# Autodesk Inventor assembly: 足全体_temp
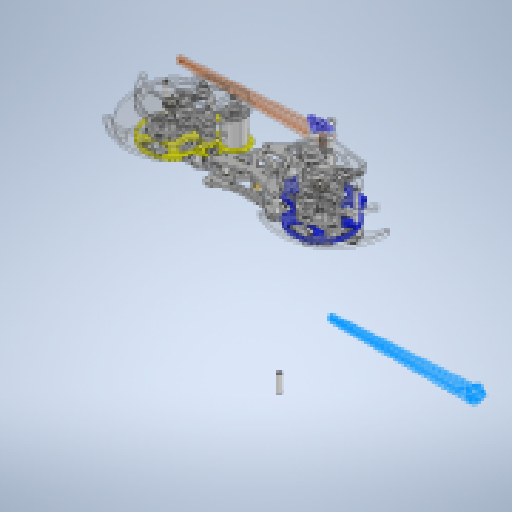
[picture p0: Inventor's stored thumbnail of the model, 512x512]
Saved by Autodesk Inventor 2023 (Build 270158000, 158)
## iProperties
Created: 2022-01-30
Part Number: 足全体_temp
Document SubType Name: Assembly
Designer: acps
Mass: 829.486 g
Surface Area: 2792.29 cm^2
Volume: 320.905 cm^3
Density: 2.58483 g/cm^3
Author: acps
## Documents named in this file (18)
- C:\Users\daphb\Documents\dabb\srdc_2\脚\足全体_temp.iam
- C:\Users\daphb\Documents\dabb\srdc_2\脚\足ユニット.iam
- C:\Users\daphb\Documents\dabb\srdc_2\スペーサ\l23.ipt
- C:\Users\daphb\Documents\dabb\srdc_2\タミヤダンパー1.iam
- C:\Users\daphb\Documents\dabb\srdc_2\スペーサ\l10.ipt
- C:\Users\daphb\Documents\dabb\srdc_2\脚\中間ユニット内_MIR1.ipt
- C:\Users\daphb\Documents\dabb\srdc_2\脚\中間ユニット外(shin).ipt
- C:\Users\daphb\Documents\dabb\srdc_2\脚\ミラー\足ユニット_MIR.iam
- C:\Users\daphb\Documents\dabb\srdc_2\脚\ミラー\l10_MIR.ipt
- C:\Users\daphb\Documents\dabb\srdc_2\脚\ミラー\l7_MIR.ipt
- C:\Users\daphb\Documents\dabb\srdc_2\スペーサ\l23_peak.ipt
- C:\Users\daphb\Documents\dabb\srdc_2\脚\ウィング関連\足 横wing固定用外フレーム.ipt
- C:\Users\daphb\Documents\dabb\srdc_2\脚\ウィング関連\足 横wing下板 .ipt
- C:\Users\daphb\Documents\dabb\srdc_2\スペーサ\l30.ipt
- C:\Users\daphb\Documents\dabb\srdc_2\スペーサ\l3.ipt
- C:\Users\daphb\Documents\dabb\srdc_2\スペーサ\l12.ipt
- C:\Users\daphb\Documents\dabb\srdc_2\脚\ウィング関連\横wing 押さえ.ipt
- C:\Users\daphb\Documents\dabb\srdc_2\脚\ウィング関連\横wing .ipt
## Components (32 placed, 17 different names)
1. 足ユニット:1 [sub-assembly] — 挿入:23, メイト:10, 挿入:35
2. l23:1
3. l23:2
4. l23:3 — 挿入:33
5. l23:4 — メイト:10, 挿入:34
6. l23:5
7. l23:6 — 挿入:21
8. l23:7
9. l23:8 — メイト:5, 挿入:31, 挿入:32
10. タミヤダンパー1:1 [sub-assembly] — 挿入:24, メイト:11
11. l10:1 — 挿入:23, 挿入:24
12. 中間ユニット外(shin):1 — メイト:5, 挿入:21, メイト:9, 挿入:32, 挿入:33, 挿入:34, 挿入:35, 挿入:45, 挿入:46, 挿入:47
13. 足ユニット_MIR:1 [sub-assembly] — 挿入:27
14. l10_MIR:1 — 挿入:27, メイト:8, 挿入:30
15. l7_MIR:1
16. タミヤダンパー1:2 [sub-assembly] — メイト:8, 挿入:30
17. 中間ユニット内_MIR1:2 — メイト:9, 挿入:31, メイト:11, 挿入:36, 挿入:37, 挿入:38, フラッシュ:1, メイト:12, メイト:13
18. l23_peak:1 — 挿入:37
19. l23_peak:2 — 挿入:36
20. l23_peak:3 — 挿入:38
21. 足 横wing固定用外フレーム:1 — メイト:14, 挿入:48
22. 足 横wing下板 :1 — フラッシュ:1, メイト:12, メイト:13, 挿入:49, 挿入:50, メイト:18
23. l30:1 — 挿入:44, 挿入:46
24. l30:2 — 挿入:42, 挿入:45
25. l30:3 — 挿入:43, 挿入:47
26. l3:1 — 挿入:42, メイト:14
27. l3:2 — 挿入:43
28. l3:3 — 挿入:44, 挿入:48
29. l12:1 — 挿入:50, 挿入:51, メイト:17
30. l12:2 — 挿入:49, メイト:15
31. 横wing 押さえ:1 — メイト:15, 挿入:51, メイト:16
32. 横wing :1 — メイト:16, メイト:17, メイト:18
## Relationships (36: Insert 23, Mate 12, Flush 1)
- メイト:5 [Mate]: l23:8 ↔ 中間ユニット外(shin):1
- 挿入:21 [Insert]: l23:6 ↔ 中間ユニット外(shin):1
- 挿入:23 [Insert]: 足ユニット:1 ↔ l10:1
- 挿入:24 [Insert]: タミヤダンパー1:1 ↔ l10:1
- 挿入:27 [Insert]: 足ユニット_MIR:1 ↔ l10_MIR:1
- メイト:8 [Mate]: l10_MIR:1 ↔ タミヤダンパー1:2
- 挿入:30 [Insert]: l10_MIR:1 ↔ タミヤダンパー1:2
- メイト:9 [Mate]: 中間ユニット外(shin):1 ↔ 中間ユニット内_MIR1:2
- 挿入:31 [Insert]: l23:8 ↔ 中間ユニット内_MIR1:2
- 挿入:32 [Insert]: l23:8 ↔ 中間ユニット外(shin):1
- 挿入:33 [Insert]: l23:3 ↔ 中間ユニット外(shin):1
- メイト:10 [Mate]: 足ユニット:1 ↔ l23:4
- 挿入:34 [Insert]: l23:4 ↔ 中間ユニット外(shin):1
- 挿入:35 [Insert] (0.5 mm): 足ユニット:1 ↔ 中間ユニット外(shin):1
- メイト:11 [Mate]: タミヤダンパー1:1 ↔ 中間ユニット内_MIR1:2
- 挿入:36 [Insert]: 中間ユニット内_MIR1:2 ↔ l23_peak:2
- 挿入:37 [Insert]: 中間ユニット内_MIR1:2 ↔ l23_peak:1
- 挿入:38 [Insert]: 中間ユニット内_MIR1:2 ↔ l23_peak:3
- フラッシュ:1 [Flush]: 中間ユニット内_MIR1:2 ↔ 足 横wing下板 :1
- メイト:12 [Mate]: 中間ユニット内_MIR1:2 ↔ 足 横wing下板 :1
- メイト:13 [Mate]: 中間ユニット内_MIR1:2 ↔ 足 横wing下板 :1
- 挿入:42 [Insert]: l30:2 ↔ l3:1
- 挿入:43 [Insert]: l30:3 ↔ l3:2
- 挿入:44 [Insert]: l30:1 ↔ l3:3
- 挿入:45 [Insert]: 中間ユニット外(shin):1 ↔ l30:2
- 挿入:46 [Insert]: 中間ユニット外(shin):1 ↔ l30:1
- 挿入:47 [Insert]: 中間ユニット外(shin):1 ↔ l30:3
- メイト:14 [Mate]: 足 横wing固定用外フレーム:1 ↔ l3:1
- 挿入:48 [Insert]: 足 横wing固定用外フレーム:1 ↔ l3:3
- 挿入:49 [Insert]: 足 横wing下板 :1 ↔ l12:2
- 挿入:50 [Insert]: 足 横wing下板 :1 ↔ l12:1
- メイト:15 [Mate]: l12:2 ↔ 横wing 押さえ:1
- 挿入:51 [Insert]: l12:1 ↔ 横wing 押さえ:1
- メイト:16 [Mate]: 横wing 押さえ:1 ↔ 横wing :1
- メイト:17 [Mate]: l12:1 ↔ 横wing :1
- メイト:18 [Mate] (5 mm): 足 横wing下板 :1 ↔ 横wing :1
